# Autodesk Inventor assembly: XL200
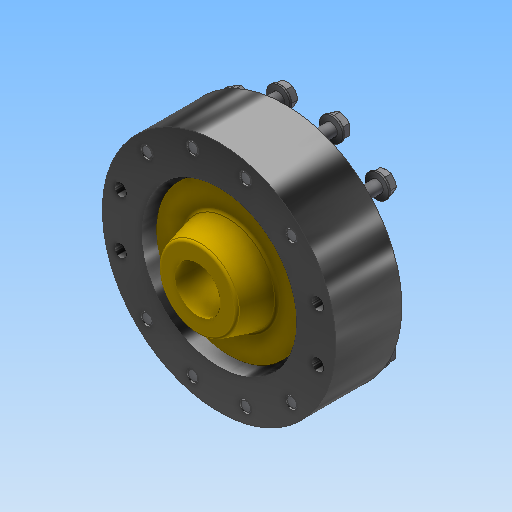
[picture p0: Inventor's stored thumbnail of the model, 512x512]
Saved by Autodesk Inventor 2020.1 (Build 241239000, 239)
## iProperties
Created: 2001-03-07
Part Number: XL200
Document SubType Name: Assembly
Designer: Joe M
Engineer: Joe M
Control State: 0
Master: False
Checked Out: False
Shininess: 20.0
Length Units: 11269
Angle Units: 11279
Time Units: 11290
Mass Units: 11283
Length Display Precision: 3
Angle Display Precision: 2
Compacted: True
Density: 0.0
Volumn: 0.0
Area: 0.0
PropertySet Name: Model Information
Author: Joe M
## Documents named in this file (6)
- C:\Users\thomastremblay\Desktop\Inventor ACP Data\Assemblies\XL200.iam
- C:\Users\thomastremblay\Desktop\Inventor ACP Data\Content Center\XL200 PART1.ipt
- C:\Users\thomastremblay\Desktop\Inventor ACP Data\Content Center\XL200 PART2.ipt
- C:\Users\thomastremblay\Desktop\Inventor ACP Data\Content Center\XL200 HEXAGON HEAD SCREW - M10 X 16 - BS 3692_1.ipt
- C:\Users\thomastremblay\Desktop\Inventor ACP Data\Content Center\MyStandard.DIN.18.81.1.ipt
- C:\Users\thomastremblay\Desktop\Inventor ACP Data\Content Center\MyStandard.DIN.162.250.1.ipt
## Components (19 placed, 5 different names)
1. PART1_1 — Flush:1, Mate:1, Mate:2, Angle:1, Insert:1
2. PART2_1 — Flush:1
3. HEXAGON HEAD SCREW - M10 X 16 - BS 3692_1_1 — Mate:1, Mate:2, Angle:1
4. DIN 931-1  (Regelgewinde) - ersetzt durch DIN EN 24 014 M12 x 90:1 — Insert:2
5. DIN 125-1  B B 13:1 — Insert:1, Insert:2
6. DIN 931-1  (Regelgewinde) - ersetzt durch DIN EN 24 014 M12 x 90:2
7. DIN 125-1  B B 13:2
8. DIN 931-1  (Regelgewinde) - ersetzt durch DIN EN 24 014 M12 x 90:3
9. DIN 125-1  B B 13:3
10. DIN 931-1  (Regelgewinde) - ersetzt durch DIN EN 24 014 M12 x 90:6
11. DIN 125-1  B B 13:6
12. DIN 931-1  (Regelgewinde) - ersetzt durch DIN EN 24 014 M12 x 90:7
13. DIN 125-1  B B 13:7
14. DIN 931-1  (Regelgewinde) - ersetzt durch DIN EN 24 014 M12 x 90:8
15. DIN 125-1  B B 13:8
16. DIN 931-1  (Regelgewinde) - ersetzt durch DIN EN 24 014 M12 x 90:9
17. DIN 125-1  B B 13:9
18. DIN 931-1  (Regelgewinde) - ersetzt durch DIN EN 24 014 M12 x 90:12
19. DIN 125-1  B B 13:12
## Component patterns: (12 elements, first: DIN 931-1  (Regelgewinde) - ersetzt durch DIN EN 24 014 M12 x 90:1 + DIN 125-1  B B 13:1)
## Relationships (6: Mate 2, Insert 2, Flush 1, Angle 1)
- Flush:1 (22 mm): PART1_1 ↔ PART2_1
- Mate:1: PART1_1 ↔ HEXAGON HEAD SCREW - M10 X 16 - BS 3692_1_1
- Mate:2: PART1_1 ↔ HEXAGON HEAD SCREW - M10 X 16 - BS 3692_1_1
- Angle:1 (0 deg): PART1_1 ↔ HEXAGON HEAD SCREW - M10 X 16 - BS 3692_1_1
- Insert:1 (20 mm): PART1_1 ↔ DIN 125-1  B B 13:1
- Insert:2: DIN 931-1  (Regelgewinde) - ersetzt durch DIN EN 24 014 M12 x 90:1 ↔ DIN 125-1  B B 13:1
